# Autodesk Inventor assembly: Welle
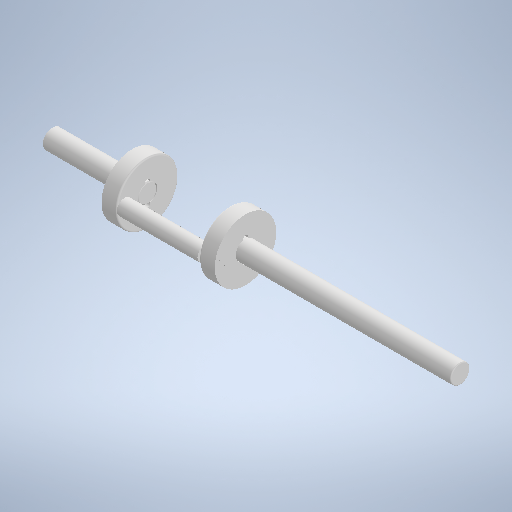
[picture p0: Inventor's stored thumbnail of the model, 512x512]
Saved by Autodesk Inventor 2025.1 (Build 291241000, 241)
## iProperties
Created: 2024-09-19
Part Number: Welle
Document SubType Name: Assembly
Designer: ffogue
Author: ffogue
## Documents named in this file (5)
- C:\Users\ffogue\Documents\Inventor\Cylinder Radial Steam Engine\Welle.iam
- C:\Users\ffogue\Documents\Inventor\Cylinder Radial Steam Engine\45.ipt
- C:\Users\ffogue\Documents\Inventor\Cylinder Radial Steam Engine\10.ipt
- C:\Users\ffogue\Documents\Inventor\Cylinder Radial Steam Engine\46.ipt
- C:\Users\ffogue\Documents\Inventor\Cylinder Radial Steam Engine\10B.ipt
## Components (5 placed, 4 different names)
1. 45:1 — Mate:1, Mate:5, Flush:2, Mate:7, Insert:1
2. 45:3 — Mate:1, Mate:2, Flush:1, Flush:3
3. 10:1 — Mate:2, Flush:1, Mate:6
4. 10B:1 — Mate:5, Flush:2, Mate:6
5. 46:2 — Mate:7, Insert:1, Flush:3
## Relationships (9: Mate 5, Flush 3, Insert 1)
- Mate:1: 45:1 ↔ 45:3
- Mate:2: 45:3 ↔ 10:1
- Flush:1: 45:3 ↔ 10:1
- Mate:5: 45:1 ↔ 10B:1
- Flush:2: 45:1 ↔ 10B:1
- Mate:6: 10:1 ↔ 10B:1
- Mate:7: 45:1 ↔ 46:2
- Insert:1: 45:1 ↔ 46:2
- Flush:3: 45:3 ↔ 46:2
